# Autodesk Inventor assembly: Assembly ebeam heater IS v0
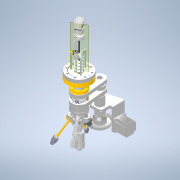
[picture p0: Inventor's stored thumbnail of the model, 180x180]
Saved by Autodesk Inventor 2020 (Build 240168000, 168)
## iProperties
Created: 2019-05-26
Part Number: Assembly ebeam heater IS v0
Document SubType Name: Assembly
Designer: isadmin
Mass: 1360.95 g
Surface Area: 5412.04 cm^2
Volume: 1345.69 cm^3
Density: 1.01134 g/cm^3
Author: isadmin
## Documents named in this file (36)
- C:\Users\ColinP\Documents\Inventor\igor\Assembly ebeam heater IS v0.iam
- Assembly ebeam heater IS v0.iam
- C:\Users\ColinP\Documents\Inventor\igor\block.ipt
- C:\Users\ColinP\Documents\Inventor\igor\Shutter.ipt
- C:\Users\ColinP\Documents\Inventor\igor\ceramic washer.ipt
- C:\Users\ColinP\Documents\Inventor\igor\Shielding.ipt
- C:\Users\ColinP\Documents\Inventor\igor\Bullet_v5_SiliconeSample.ipt
- C:\Users\ColinP\Documents\Inventor\igor\Bullet_v5_SiliconeSample_TopPart.ipt
- C:\Users\ColinP\Documents\Inventor\igor\670000.ipt
- C:\Users\ColinP\Documents\Inventor\igor\MCF275-FlgMplxr-Cr1A5_(53-321020-A).ipt
- C:\Users\ColinP\Documents\Inventor\igor\665501.ipt
- C:\Users\ColinP\Documents\Inventor\igor\rotatable rod table.ipt
- C:\Users\ColinP\Documents\Inventor\igor\updated table+legs.iam
- C:\Users\ColinP\Documents\Inventor\igor\square eyelet.ipt
- C:\Users\ColinP\Documents\Inventor\igor\buffer.ipt
- C:\Users\ColinP\Documents\Inventor\igor\4.5to2.75converotr.ipt
- C:\Users\ColinP\Documents\Inventor\igor\rotaryconnector.ipt
- C:\Users\ColinP\Documents\Inventor\igor\140007.ipt
- C:\Users\ColinP\Documents\Inventor\Content Center Files\R2020\en-US\ISO 4029\ISO 4029 - M2 x 2 - ISO.ipt
- C:\Users\ColinP\Documents\Inventor\igor\9312007.iam
- C:\Users\ColinP\Documents\Inventor\igor\eft0181032.ipt
- C:\Users\ColinP\Documents\Inventor\igor\filwasher.ipt
- C:\Users\ColinP\Documents\Inventor\igor\filament.ipt
- C:\Users\ColinP\Documents\Inventor\igor\fileholddub.ipt
- C:\Users\ColinP\Documents\Inventor\Content Center Files\R2020\en-US\ISO 4017(1)\ISO 4017 - M2.5 x 5 - ISO.ipt
- C:\Users\ColinP\Documents\Inventor\igor\flange 4_5 double_sided.ipt
- C:\Users\ColinP\Downloads\98401A910_18-8 STAINLESS STEEL COTTER PIN.ipt
- C:\Users\ColinP\Documents\Inventor\igor\water.ipt
- C:\Users\ColinP\Downloads\610003 rev A.ipt
- C:\Users\ColinP\Documents\Inventor\igor\waterpipe.ipt
- C:\Users\ColinP\Downloads\SS-4-VCR-3-4MTW-SwagelokCompany-07-18-2019.ipt
- C:\Users\ColinP\Downloads\SS-4-VCR-7-4-SwagelokCompany-07-18-2019.ipt
- C:\Users\ColinP\Downloads\SS-4-VCO-7-4-SwagelokCompany-07-19-2019.ipt
- C:\Users\ColinP\Documents\Inventor\igor\undertable.ipt
- C:\Users\ColinP\Documents\Inventor\igor\stability copy2.ipt
- C:\Users\ColinP\Documents\Inventor\igor\stability copy.ipt
## Components (118 placed, 34 different names)
1. rotatable rod table:1 — Mate:48, Insert:171, Insert:173, Insert:174, Insert:175, Rigid:18, Insert:176, Insert:177, Insert:181, Mate:101, Insert:183, Insert:187, Mate:205, Mate:232, Mate:234
2. block for bullet:1
3. Shutter:1
4. ceramic washer:1
5. ceramic washer:2
6. ceramic washer:3
7. ceramic washer:4
8. Shielding:1
9. ceramic washer:5
10. ceramic washer:6
11. ceramic washer:7
12. ceramic washer:8
13. Bullet_v5_SiliconeSample:1
14. Bullet_v5_SiliconeSample_TopPart:1
15. rotation_670000:1 — Rotational:3, Rigid:18
16. MCF275-FlgMplxr-Cr1A5_(53-321020-A):1 — Rotational:3, Rigid:5, Rigid:19, Rotational:10, Rotational:11, Rigid:20
17. zstage_665501:1 — Rigid:8, Cylindrical:1, Mate:235
18. 140007:1 — Rigid:5, Rigid:8, Insert:131, Insert:132, Insert:133, Insert:134, Insert:135, Insert:136
19. updated table+legs:1 [sub-assembly] — Mate:48, Mate:72, Rigid:14, Insert:166, Angle:1, Mate:107, Mate:108, Mate:109, Mate:110, Mate:111, Mate:115, Mate:116, Mate:117, Mate:119, Mate:120, Mate:121, Mate:122, Mate:123, Mate:124, Mate:125, Mate:137, Mate:140, Mate:141, Mate:189, Mate:190, Mate:191, Mate:200, Mate:201, Mate:202, Mate:213, Mate:215, Mate:216, Mate:217, Mate:218, Mate:219, Mate:220, Rotational:12, Rigid:22, Mate:233
20. buffer:4 — Insert:173
21. square eyelet:24
22. square eyelet:25 — Mate:218
23. square eyelet:26
24. buffer:5 — Insert:171
25. square eyelet:27
26. square eyelet:28 — Mate:216
27. square eyelet:29
28. buffer:6 — Insert:161, Insert:162, Insert:163, Insert:174
29. buffer:7 — Insert:176
30. square eyelet:33
31. square eyelet:34 — Mate:220
32. square eyelet:35
33. buffer:9 — Insert:177
34. square eyelet:39
35. square eyelet:40 — Mate:217
36. square eyelet:41
37. rotaryconnector:2 — Insert:149, Insert:150, Insert:151, Insert:152, Insert:187
38. 4.5to2.75converotr:1 — Rigid:21, Cylindrical:1, Mate:235
39. square eyelet:49 — Insert:134
40. square eyelet:50 — Insert:135
41. square eyelet:51 — Insert:133
42. square eyelet:52 — Insert:131, Mate:72
43. square eyelet:53 — Insert:132
44. square eyelet:54 — Insert:136
45. buffer:10 — Insert:175
46. square eyelet:55 — Mate:215
47. square eyelet:56
48. square eyelet:57
49. 9312007:1 [sub-assembly] — Rigid:19
50. eft0181032:1 — Rigid:20
51. square eyelet:64 — Insert:162
52. square eyelet:65 — Insert:163
53. square eyelet:66 — Insert:161, Mate:219
54. filament:1 — Mate:126, Mate:127
55. filwasher:2 — Rigid:14, Insert:168, Mate:206, Rotational:12
56. fileholddub:1 — Insert:166, Rigid:17, Rotational:9, Angle:1
57. filwasher:5 — Rotational:9, Insert:169, Mate:207
58. filwasher:6 — Rigid:17, Insert:170, Mate:127
59. filwasher:7 — Insert:167, Mate:126, Rigid:22
60. buffer:11 — Insert:178, Insert:179, Insert:180, Insert:181, Mate:214, Insert:199, Insert:200
61. square eyelet:67 — Insert:178
62. square eyelet:68 — Insert:179
63. square eyelet:69 — Insert:180
64. flange 4_5 double_sided:1 — Mate:101, Rigid:21, Insert:196, Insert:197, Insert:198
65. ISO 4029 M2 x 2:1 — Insert:152
66. ISO 4029 M2 x 2:2 — Insert:150
67. ISO 4029 M2 x 2:3 — Insert:151
68. ISO 4029 M2 x 2:4 — Insert:149
69. ISO 4017 M2.5 x 5:1 — Insert:167
70. ISO 4017 M2.5 x 5:2 — Insert:168
71. ISO 4017 M2.5 x 5:3 — Insert:169
72. ISO 4017 M2.5 x 5:4 — Insert:170
73. 98401A910_18-8 STAINLESS STEEL COTTER PIN:1 — Mate:108
74. 98401A910_18-8 STAINLESS STEEL COTTER PIN:2 — Mate:109
75. 98401A910_18-8 STAINLESS STEEL COTTER PIN:3 — Mate:107
76. 98401A910_18-8 STAINLESS STEEL COTTER PIN:4 — Mate:111
77. 98401A910_18-8 STAINLESS STEEL COTTER PIN:5 — Mate:137
78. 98401A910_18-8 STAINLESS STEEL COTTER PIN:6 — Mate:110
79. 98401A910_18-8 STAINLESS STEEL COTTER PIN:7 — Mate:140
80. 98401A910_18-8 STAINLESS STEEL COTTER PIN:8 — Mate:116
81. 98401A910_18-8 STAINLESS STEEL COTTER PIN:9 — Mate:115
82. 98401A910_18-8 STAINLESS STEEL COTTER PIN:10 — Mate:117
83. 98401A910_18-8 STAINLESS STEEL COTTER PIN:11 — Mate:119
84. 98401A910_18-8 STAINLESS STEEL COTTER PIN:12 — Mate:141
85. 98401A910_18-8 STAINLESS STEEL COTTER PIN:13 — Mate:121
86. 98401A910_18-8 STAINLESS STEEL COTTER PIN:14 — Mate:122
87. 98401A910_18-8 STAINLESS STEEL COTTER PIN:15 — Mate:120
88. 98401A910_18-8 STAINLESS STEEL COTTER PIN:16 — Mate:123
89. 98401A910_18-8 STAINLESS STEEL COTTER PIN:17 — Mate:125
90. 98401A910_18-8 STAINLESS STEEL COTTER PIN:18 — Mate:124
91. water:1 — Insert:183, Insert:188, Insert:189, Insert:190, Mate:213, Mate:214
92. square eyelet:70 — Insert:190
93. square eyelet:71 — Insert:189
94. square eyelet:72 — Insert:188
95. 610003 rev A:1 — Mate:175, Mate:176, Mate:178, Rotational:10, Mate:196, Mate:197
96. 610003 rev A:2 — Mate:181, Mate:182, Mate:184, Mate:186, Rotational:11, Mate:195, Mate:198
97. SS-4-VCR-3-4MTW-SwagelokCompany-07-18-2019:1 — Mate:175, Mate:176, Mate:177, Mate:188
98. SS-4-VCR-3-4MTW-SwagelokCompany-07-18-2019:2 — Mate:177, Mate:178, Mate:179
99. SS-4-VCR-7-4-SwagelokCompany-07-18-2019:1 — Mate:179, Mate:188
100. SS-4-VCR-3-4MTW-SwagelokCompany-07-18-2019:3 — Mate:181, Mate:182, Mate:183, Mate:187
101. SS-4-VCR-3-4MTW-SwagelokCompany-07-18-2019:4 — Mate:183, Mate:184, Mate:185
102. SS-4-VCR-7-4-SwagelokCompany-07-18-2019:2 — Mate:185, Mate:186, Mate:187
103. 98401A910_18-8 STAINLESS STEEL COTTER PIN:22 — Mate:189
104. 98401A910_18-8 STAINLESS STEEL COTTER PIN:23 — Mate:191
105. 98401A910_18-8 STAINLESS STEEL COTTER PIN:24 — Mate:190
106. SS-4-VCO-7-4-SwagelokCompany-07-19-2019:1 — Mate:195, Mate:198
107. SS-4-VCO-7-4-SwagelokCompany-07-19-2019:2 — Mate:196, Mate:197
108. 98401A910_18-8 STAINLESS STEEL COTTER PIN:25 — Mate:201
109. 98401A910_18-8 STAINLESS STEEL COTTER PIN:26 — Mate:200
110. 98401A910_18-8 STAINLESS STEEL COTTER PIN:27 — Mate:202
111. filament:2 — Mate:206, Mate:207
112. waterpipe:1 — Insert:200
113. waterpipe:2 — Insert:199
114. undertable:1 — Mate:232, Mate:233
115. stability copy2:1 — Insert:193, Insert:198
116. stability copy2:2 — Insert:194, Insert:197
117. stability copy2:3 — Insert:195, Insert:196
118. stability copy:1 — Mate:234, Insert:193, Insert:194, Insert:195
## Relationships (160: Mate 83, Insert 59, WeldJoint 9, RevoluteJoint 5, Flush 2, Angle 1, CylindricalJoint 1)
- [Mate]: block for bullet:1 ↔ Shutter:1
- [Mate]: block for bullet:1 ↔ Shutter:1
- [Mate]: block for bullet:1 ↔ Shutter:1
- [Mate]: block for bullet:1 ↔ ceramic washer:2
- [Mate]: block for bullet:1 ↔ ceramic washer:2
- [Mate]: block for bullet:1 ↔ ceramic washer:1
- [Mate]: block for bullet:1 ↔ ceramic washer:1
- [Mate]: block for bullet:1 ↔ ceramic washer:4
- [Mate]: block for bullet:1 ↔ ceramic washer:4
- [Mate]: block for bullet:1 ↔ ceramic washer:3
- [Mate]: block for bullet:1 ↔ ceramic washer:3
- [Mate]: ceramic washer:1 ↔ Shielding:1
- [Flush]: block for bullet:1 ↔ Shielding:1
- [Flush]: block for bullet:1 ↔ Shielding:1
- [Mate]: block for bullet:1 ↔ ceramic washer:5
- [Mate]: block for bullet:1 ↔ ceramic washer:5
- [Mate]: block for bullet:1 ↔ ceramic washer:6
- [Mate]: block for bullet:1 ↔ ceramic washer:6
- [Mate]: block for bullet:1 ↔ ceramic washer:7
- [Mate]: block for bullet:1 ↔ ceramic washer:7
- [Mate]: block for bullet:1 ↔ ceramic washer:8
- [Mate]: block for bullet:1 ↔ ceramic washer:8
- [Mate] (0.0254 mm): Bullet_v5_SiliconeSample:1 ↔ Bullet_v5_SiliconeSample_TopPart:1
- [Mate]: Bullet_v5_SiliconeSample:1 ↔ Bullet_v5_SiliconeSample_TopPart:1
- [Insert]: block for bullet:1 ↔ Bullet_v5_SiliconeSample:1
- [Insert]: rotatable rod table:1 ↔ block for bullet:1
- [Insert]: rotatable rod table:1 ↔ block for bullet:1
- [Insert]: buffer:4 ↔ square eyelet:25
- [Insert]: buffer:4 ↔ square eyelet:24
- [Insert]: buffer:4 ↔ square eyelet:26
- [Insert]: buffer:5 ↔ square eyelet:28
- [Insert]: buffer:5 ↔ square eyelet:27
- [Insert]: buffer:5 ↔ square eyelet:29
- [Insert]: buffer:7 ↔ square eyelet:34
- [Insert]: buffer:7 ↔ square eyelet:33
- [Insert]: buffer:7 ↔ square eyelet:35
- [Insert]: buffer:9 ↔ square eyelet:40
- [Insert]: buffer:9 ↔ square eyelet:39
- [Insert]: buffer:9 ↔ square eyelet:41
- Mate:48: rotatable rod table:1 ↔ updated table+legs:1
- Rotational:3 [RevoluteJoint]: rotation_670000:1 ↔ MCF275-FlgMplxr-Cr1A5_(53-321020-A):1
- Rigid:5 [WeldJoint]: MCF275-FlgMplxr-Cr1A5_(53-321020-A):1 ↔ 140007:1
- Rigid:8 [WeldJoint]: zstage_665501:1 ↔ 140007:1
- Insert:131: 140007:1 ↔ square eyelet:52
- Insert:132: 140007:1 ↔ square eyelet:53
- Insert:133: 140007:1 ↔ square eyelet:51
- Insert:134: 140007:1 ↔ square eyelet:49
- Insert:135: 140007:1 ↔ square eyelet:50
- Insert:136: 140007:1 ↔ square eyelet:54
- [Insert]: buffer:10 ↔ square eyelet:56
- [Insert]: buffer:10 ↔ square eyelet:55
- [Insert]: buffer:10 ↔ square eyelet:57
- Insert:149: rotaryconnector:2 ↔ ISO 4029 M2 x 2:4
- Insert:150: rotaryconnector:2 ↔ ISO 4029 M2 x 2:2
- Insert:151: rotaryconnector:2 ↔ ISO 4029 M2 x 2:3
- Insert:152: rotaryconnector:2 ↔ ISO 4029 M2 x 2:1
- Rigid:19 [WeldJoint]: MCF275-FlgMplxr-Cr1A5_(53-321020-A):1 ↔ 9312007:1
- Mate:72: updated table+legs:1 ↔ square eyelet:52
- Insert:161: buffer:6 ↔ square eyelet:66
- Insert:162: buffer:6 ↔ square eyelet:64
- Insert:163: buffer:6 ↔ square eyelet:65
- Rigid:14 [WeldJoint]: updated table+legs:1 ↔ filwasher:2
- Insert:166 (-7.62 mm): updated table+legs:1 ↔ fileholddub:1
- Rigid:17 [WeldJoint]: fileholddub:1 ↔ filwasher:6
- Rotational:9 [RevoluteJoint]: fileholddub:1 ↔ filwasher:5
- Insert:167: filwasher:7 ↔ ISO 4017 M2.5 x 5:1
- Insert:168: filwasher:2 ↔ ISO 4017 M2.5 x 5:2
- Insert:169: filwasher:5 ↔ ISO 4017 M2.5 x 5:3
- Insert:170: filwasher:6 ↔ ISO 4017 M2.5 x 5:4
- Insert:171 (165.1 mm): rotatable rod table:1 ↔ buffer:5
- Insert:173 (203.2 mm): rotatable rod table:1 ↔ buffer:4
- Insert:174 (228.6 mm): rotatable rod table:1 ↔ buffer:6
- Insert:175 (152.4 mm): rotatable rod table:1 ↔ buffer:10
- Angle:1 (180 deg): updated table+legs:1 ↔ fileholddub:1
- Rigid:18 [WeldJoint]: rotatable rod table:1 ↔ rotation_670000:1
- Insert:176 (241.3 mm): rotatable rod table:1 ↔ buffer:7
- Insert:177 (177.8 mm): rotatable rod table:1 ↔ buffer:9
- Insert:178: buffer:11 ↔ square eyelet:67
- Insert:179: buffer:11 ↔ square eyelet:68
- Insert:180: buffer:11 ↔ square eyelet:69
- Insert:181 (139.7 mm): rotatable rod table:1 ↔ buffer:11
- Mate:101: rotatable rod table:1 ↔ flange 4_5 double_sided:1
- Mate:107: updated table+legs:1 ↔ 98401A910_18-8 STAINLESS STEEL COTTER PIN:3
- Mate:108: updated table+legs:1 ↔ 98401A910_18-8 STAINLESS STEEL COTTER PIN:1
- Mate:109: updated table+legs:1 ↔ 98401A910_18-8 STAINLESS STEEL COTTER PIN:2
- Mate:110: updated table+legs:1 ↔ 98401A910_18-8 STAINLESS STEEL COTTER PIN:6
- Mate:111: updated table+legs:1 ↔ 98401A910_18-8 STAINLESS STEEL COTTER PIN:4
- Mate:115: updated table+legs:1 ↔ 98401A910_18-8 STAINLESS STEEL COTTER PIN:9
- Mate:116: updated table+legs:1 ↔ 98401A910_18-8 STAINLESS STEEL COTTER PIN:8
- Mate:117: updated table+legs:1 ↔ 98401A910_18-8 STAINLESS STEEL COTTER PIN:10
- Mate:119: updated table+legs:1 ↔ 98401A910_18-8 STAINLESS STEEL COTTER PIN:11
- Mate:120: updated table+legs:1 ↔ 98401A910_18-8 STAINLESS STEEL COTTER PIN:15
- Mate:121: updated table+legs:1 ↔ 98401A910_18-8 STAINLESS STEEL COTTER PIN:13
- Mate:122: updated table+legs:1 ↔ 98401A910_18-8 STAINLESS STEEL COTTER PIN:14
- Mate:123: updated table+legs:1 ↔ 98401A910_18-8 STAINLESS STEEL COTTER PIN:16
- Mate:124: updated table+legs:1 ↔ 98401A910_18-8 STAINLESS STEEL COTTER PIN:18
- Mate:125: updated table+legs:1 ↔ 98401A910_18-8 STAINLESS STEEL COTTER PIN:17
- Mate:126: filament:1 ↔ filwasher:7
- Mate:127: filament:1 ↔ filwasher:6
- Insert:183 (34.29 mm): rotatable rod table:1 ↔ water:1
- Mate:137: updated table+legs:1 ↔ 98401A910_18-8 STAINLESS STEEL COTTER PIN:5
- Mate:140: updated table+legs:1 ↔ 98401A910_18-8 STAINLESS STEEL COTTER PIN:7
- Mate:141: updated table+legs:1 ↔ 98401A910_18-8 STAINLESS STEEL COTTER PIN:12
- Mate:175: 610003 rev A:1 ↔ SS-4-VCR-3-4MTW-SwagelokCompany-07-18-2019:1
- Mate:176: 610003 rev A:1 ↔ SS-4-VCR-3-4MTW-SwagelokCompany-07-18-2019:1
- Mate:177: SS-4-VCR-3-4MTW-SwagelokCompany-07-18-2019:1 ↔ SS-4-VCR-3-4MTW-SwagelokCompany-07-18-2019:2
- Mate:178: 610003 rev A:1 ↔ SS-4-VCR-3-4MTW-SwagelokCompany-07-18-2019:2
- Mate:179: SS-4-VCR-3-4MTW-SwagelokCompany-07-18-2019:2 ↔ SS-4-VCR-7-4-SwagelokCompany-07-18-2019:1
- Rotational:10 [RevoluteJoint]: MCF275-FlgMplxr-Cr1A5_(53-321020-A):1 ↔ 610003 rev A:1
- Mate:181: 610003 rev A:2 ↔ SS-4-VCR-3-4MTW-SwagelokCompany-07-18-2019:3
- Mate:182: 610003 rev A:2 ↔ SS-4-VCR-3-4MTW-SwagelokCompany-07-18-2019:3
- Mate:183: SS-4-VCR-3-4MTW-SwagelokCompany-07-18-2019:3 ↔ SS-4-VCR-3-4MTW-SwagelokCompany-07-18-2019:4
- Mate:184: 610003 rev A:2 ↔ SS-4-VCR-3-4MTW-SwagelokCompany-07-18-2019:4
- Mate:185: SS-4-VCR-3-4MTW-SwagelokCompany-07-18-2019:4 ↔ SS-4-VCR-7-4-SwagelokCompany-07-18-2019:2
- Mate:186: 610003 rev A:2 ↔ SS-4-VCR-7-4-SwagelokCompany-07-18-2019:2
- Mate:187: SS-4-VCR-3-4MTW-SwagelokCompany-07-18-2019:3 ↔ SS-4-VCR-7-4-SwagelokCompany-07-18-2019:2
- Mate:188: SS-4-VCR-3-4MTW-SwagelokCompany-07-18-2019:1 ↔ SS-4-VCR-7-4-SwagelokCompany-07-18-2019:1
- Rotational:11 [RevoluteJoint]: MCF275-FlgMplxr-Cr1A5_(53-321020-A):1 ↔ 610003 rev A:2
- Mate:189: updated table+legs:1 ↔ 98401A910_18-8 STAINLESS STEEL COTTER PIN:22
- Mate:190: updated table+legs:1 ↔ 98401A910_18-8 STAINLESS STEEL COTTER PIN:24
- Mate:191: updated table+legs:1 ↔ 98401A910_18-8 STAINLESS STEEL COTTER PIN:23
- Mate:195: 610003 rev A:2 ↔ SS-4-VCO-7-4-SwagelokCompany-07-19-2019:1
- Mate:196: 610003 rev A:1 ↔ SS-4-VCO-7-4-SwagelokCompany-07-19-2019:2
- Mate:197: 610003 rev A:1 ↔ SS-4-VCO-7-4-SwagelokCompany-07-19-2019:2
- Mate:198: 610003 rev A:2 ↔ SS-4-VCO-7-4-SwagelokCompany-07-19-2019:1
- Insert:187 (-12.7 mm): rotatable rod table:1 ↔ rotaryconnector:2
- Rigid:20 [WeldJoint]: MCF275-FlgMplxr-Cr1A5_(53-321020-A):1 ↔ eft0181032:1
- Rigid:21 [WeldJoint]: 4.5to2.75converotr:1 ↔ flange 4_5 double_sided:1
- Cylindrical:1: zstage_665501:1 ↔ 4.5to2.75converotr:1
- Mate:200: updated table+legs:1 ↔ 98401A910_18-8 STAINLESS STEEL COTTER PIN:26
- Mate:201: updated table+legs:1 ↔ 98401A910_18-8 STAINLESS STEEL COTTER PIN:25
- Mate:202: updated table+legs:1 ↔ 98401A910_18-8 STAINLESS STEEL COTTER PIN:27
- Mate:205: rotatable rod table:1
- Insert:188: water:1 ↔ square eyelet:72
- Insert:189: water:1 ↔ square eyelet:71
- Insert:190: water:1 ↔ square eyelet:70
- Mate:206: filwasher:2 ↔ filament:2
- Mate:207: filwasher:5 ↔ filament:2
- Mate:213: updated table+legs:1 ↔ water:1
- Mate:214: buffer:11 ↔ water:1
- Mate:215: updated table+legs:1 ↔ square eyelet:55
- Mate:216: updated table+legs:1 ↔ square eyelet:28
- Mate:217: updated table+legs:1 ↔ square eyelet:40
- Mate:218: updated table+legs:1 ↔ square eyelet:25
- Mate:219: updated table+legs:1 ↔ square eyelet:66
- Mate:220: updated table+legs:1 ↔ square eyelet:34
- Rotational:12 [RevoluteJoint]: updated table+legs:1 ↔ filwasher:2
- Rigid:22 [WeldJoint]: updated table+legs:1 ↔ filwasher:7
- Mate:232: rotatable rod table:1 ↔ undertable:1
- Mate:233: updated table+legs:1 ↔ undertable:1
- Mate:234: rotatable rod table:1 ↔ stability copy:1
- Insert:193: stability copy2:1 ↔ stability copy:1
- Insert:194: stability copy2:2 ↔ stability copy:1
- Insert:195: stability copy2:3 ↔ stability copy:1
- Insert:196: flange 4_5 double_sided:1 ↔ stability copy2:3
- Insert:197: flange 4_5 double_sided:1 ↔ stability copy2:2
- Insert:198: flange 4_5 double_sided:1 ↔ stability copy2:1
- Mate:235: zstage_665501:1 ↔ 4.5to2.75converotr:1
- Insert:199: buffer:11 ↔ waterpipe:2
- Insert:200: buffer:11 ↔ waterpipe:1
## Named parameters: d75_d58 = 0 mm, d76_d19 = 0 mm, d77_d22_d25 = 0 mm, d78_d23_d26 = 0 mm, d79_d24_d35 = 0 mm, d80_d25_d36 = 0 mm, d81_d26_d37 = 0 mm, d82_d27_d38 = 0 mm, d83_d28_d39 = 0 mm, d84_d29_d40 = 0 mm, d85_d30_d41 = 0 mm, d86_d31_d42 = 0 mm, d87_d43 = 0 mm, d88_d44 = 0 mm, d89_d45 = 0 mm, d90_d46 = 0 mm, d91_d47 = 0 mm, d92_d48 = 0 mm, d93_d49 = 0 mm, d94_d50 = 0 mm, d95_d51 = 0 mm, d96_d52 = 0 mm, d97_d53 = 0 mm, d98_d56_d0 = 0.0254 mm, d99_d57_d1 = 0 mm, d148_d124_d114_d111 = 0 mm, d149_d125_d115_d112 = 0 mm, d150_d126_d116_d113 = 0 mm, d152_d124_d114_d111 = 0 mm, d153_d125_d115_d112 = 0 mm, d154_d126_d116_d113 = 0 mm, d163_d124_d114_d111 = 0 mm, d164_d125_d115_d112 = 0 mm, d165_d126_d116_d113 = 0 mm, d175_d111 = 0 mm, d176_d112 = 0 mm, d177_d113 = 0 mm, d314_d124_d114_d111 = 0 mm, d315_d125_d115_d112 = 0 mm, d316_d126_d116_d113 = 0 mm, sa_0 = 444.822
note: some values were not read from the file. Shown as the stored number, unit unknown: "sa_0".
